# Autodesk Inventor assembly: Ensamble
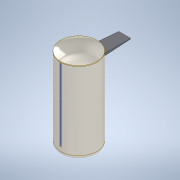
[picture p0: Inventor's stored thumbnail of the model, 180x180]
Saved by Autodesk Inventor 2020 (Build 240168000, 168)
## iProperties
Created: 2020-10-28
Part Number: Ensamble
Document SubType Name: Assembly
Designer: aaron
Author: aaron
## Documents named in this file (7)
- C:\Users\aaron\OneDrive\Escritorio\Proyecto\Ensamble.iam
- C:\Users\aaron\OneDrive\Escritorio\Proyecto\Exterior.ipt
- C:\Users\aaron\OneDrive\Escritorio\Proyecto\Deposito.iam
- C:\Users\aaron\OneDrive\Escritorio\Proyecto\Surtidor.ipt
- C:\Users\aaron\OneDrive\Escritorio\Proyecto\ConectorPTFE_4.ipt
- C:\Users\aaron\OneDrive\Escritorio\Proyecto\Electronica.iam
- C:\Users\aaron\OneDrive\Escritorio\Proyecto\Tapadera.ipt
## Components (6 placed, 6 different names)
1. Exterior:1 — Mate:1, Mate:2, Mate:3, Mate:4, Mate:5, Mate:6, Mate:7, Angle:1, Angle:2, Mate:9, Mate:11, Mate:12, Mate:13
2. Surtidor:1 — Mate:1
3. Deposito:1 [sub-assembly] — Mate:2, Mate:3, Mate:4, Mate:10
4. ConectorPTFE_4:1 — Mate:5, Mate:6
5. Electronica:1 [sub-assembly] — Angle:2, Mate:9, Mate:10, Mate:11
6. Tapadera:1 — Mate:12, Mate:13
## Relationships (14: Mate 12, Angle 2)
- Mate:1: Exterior:1 ↔ Surtidor:1
- Mate:2: Exterior:1 ↔ Deposito:1
- Mate:3: Exterior:1 ↔ Deposito:1
- Mate:4: Exterior:1 ↔ Deposito:1
- Mate:5: Exterior:1 ↔ ConectorPTFE_4:1
- Mate:6 (-41 mm): Exterior:1 ↔ ConectorPTFE_4:1
- Mate:7: Exterior:1
- Angle:1 (90 deg): Exterior:1
- Angle:2 (0 deg): Exterior:1 ↔ Electronica:1
- Mate:9: Exterior:1 ↔ Electronica:1
- Mate:10: Deposito:1 ↔ Electronica:1
- Mate:11: Exterior:1 ↔ Electronica:1
- Mate:12: Exterior:1 ↔ Tapadera:1
- Mate:13: Exterior:1 ↔ Tapadera:1
